# Autodesk Inventor assembly: 2008-FIRST-Wheel
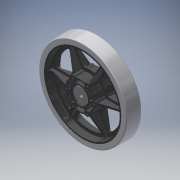
[picture p0: Inventor's stored thumbnail of the model, 180x180]
Saved by Autodesk Inventor 2018 (Build 220112000, 112)
## iProperties
Created: 2008-01-05
Part Number: 2008-FIRST-Wheel
Document SubType Name: Assembly
Designer: 21chinton
Sending System: Autodesk Inventor 11
Preprocessor: Autodesk Inventor 11
Title: E:\2008\First 08 Wheel.stp
Author: pz0s5n
## Documents named in this file (4)
- C:\Users\21chinton\Documents\GitHub\RobotDesigns2018\2008-FIRST-Wheel.iam
- C:\Users\21chinton\Downloads\Hub.ipt
- C:\Users\21chinton\Downloads\Tread.ipt
- H:\DDP\robotics\rod.5.ipt
## Components (3 placed, 3 different names)
1. Hub:1 — Mate:1
2. Tread:1
3. rod.5:1 — Mate:1
## Relationships (1: Mate 1)
- Mate:1: Hub:1 ↔ rod.5:1
